# Autodesk Inventor assembly: right_leg
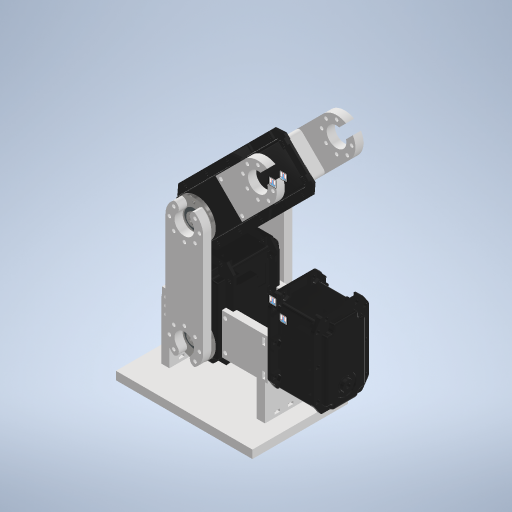
[picture p0: Inventor's stored thumbnail of the model, 512x512]
Saved by Autodesk Inventor 2024.3 (Build 283343000, 343)
## iProperties
Created: 2024-09-16
Part Number: right_leg
Document SubType Name: Assembly
Designer: USER
Author: USER
## Documents named in this file (12)
- C:\Users\USER\Desktop\로빛 예비인턴\(git)19기 이원준 격투로봇 설계파일\Lower_body\right_leg.iam
- C:\Users\USER\Desktop\로빛 예비인턴\(git)19기 이원준 격투로봇 설계파일\Lower_body\_foot.ipt
- C:\Users\USER\Desktop\로빛 예비인턴\(git)19기 이원준 격투로봇 설계파일\Lower_body\_foot_adt.ipt
- C:\Users\USER\Desktop\로빛 예비인턴\(git)19기 이원준 격투로봇 설계파일\Lower_body\_shim.ipt
- C:\Users\USER\Desktop\로빛 예비인턴\(git)19기 이원준 격투로봇 설계파일\Lower_body\_idle_adt.ipt
- C:\Users\USER\Desktop\로빛 예비인턴\(git)19기 이원준 격투로봇 설계파일\Lower_body\_adle_adt_2.ipt
- C:\Users\USER\Desktop\로빛 예비인턴\(git)19기 이원준 격투로봇 설계파일\motor\Motor_106.iam
- C:\Users\USER\Desktop\로빛 예비인턴\(git)19기 이원준 격투로봇 설계파일\아이들러\64아이들러.iam
- C:\Users\USER\Desktop\로빛 예비인턴\(git)19기 이원준 격투로봇 설계파일\motor\Motor_64_no_idle_ver.iam
- C:\Users\USER\Desktop\로빛 예비인턴\(git)19기 이원준 격투로봇 설계파일\Lower_body\_108-64_adt.ipt
- C:\Users\USER\Desktop\로빛 예비인턴\(git)19기 이원준 격투로봇 설계파일\Lower_body\_thigh.ipt
- C:\Users\USER\Desktop\로빛 예비인턴\(git)19기 이원준 격투로봇 설계파일\Lower_body\_thigh_2.ipt
## Components (18 placed, 11 different names)
1. _foot:1
2. _foot_adt:1 — 각도:2, 삽입:46, 삽입:47
3. _foot_adt:2
4. _shim:1 — 삽입:34, 삽입:36
5. _shim:2 — 삽입:35, 삽입:37, 삽입:38, 삽입:45, 각도:2
6. _idle_adt:1 — 삽입:43
7. _adle_adt_2:1
8. _idle_adt:2 — 삽입:42
9. 64아이들러:1 [sub-assembly] — 삽입:46, 삽입:47
10. Motor_64_no_idle_ver:1 [sub-assembly]
11. _108-64_adt:1 — 삽입:41
12. _108-64_adt:2 — 삽입:40
13. _thigh:1 — 삽입:31, 삽입:44
14. _thigh:2 — 삽입:29, 삽입:30, 삽입:32, 삽입:33
15. _thigh_2:1
16. _thigh_2:2
17. Motor_106:1 [sub-assembly] — 삽입:36, 삽입:37, 삽입:38, 삽입:40, 삽입:41, 삽입:42, 삽입:43
18. Motor_106:2 [sub-assembly] — 삽입:29, 삽입:30, 삽입:31, 삽입:32, 삽입:33, 삽입:34, 삽입:35, 삽입:44, 삽입:45
## Relationships (36: Insert 35, Angle 1)
- [Insert]: _foot:1 ↔ _foot_adt:1
- [Insert]: _foot:1 ↔ _foot_adt:1
- [Insert]: _foot:1 ↔ _foot_adt:2
- [Insert]: _foot:1 ↔ _foot_adt:2
- [Insert]: _adle_adt_2:1 ↔ _idle_adt:2
- [Insert]: _adle_adt_2:1 ↔ _idle_adt:2
- [Insert]: _idle_adt:1 ↔ _adle_adt_2:1
- [Insert]: _idle_adt:1 ↔ _adle_adt_2:1
- [Insert]: _foot_adt:1 ↔ 64아이들러:1
- [Insert]: _adle_adt_2:1 ↔ 64아이들러:1
- [Insert]: Motor_64_no_idle_ver:1 ↔ _108-64_adt:2
- [Insert]: Motor_64_no_idle_ver:1 ↔ _108-64_adt:2
- [Insert]: Motor_64_no_idle_ver:1 ↔ _108-64_adt:1
- [Insert]: _thigh:1 ↔ _thigh_2:1
- [Insert]: _thigh:1 ↔ _thigh_2:1
- [Insert]: _thigh:2 ↔ _thigh_2:2
- [Insert]: _thigh:2 ↔ _thigh_2:2
- 삽입:29 [Insert]: _thigh:2 ↔ Motor_106:2
- 삽입:30 [Insert]: _thigh:2 ↔ Motor_106:2
- 삽입:31 [Insert]: _thigh:1 ↔ Motor_106:2
- 삽입:32 [Insert]: _thigh:2 ↔ Motor_106:2
- 삽입:33 [Insert]: _thigh:2 ↔ Motor_106:2
- 삽입:34 [Insert]: _shim:1 ↔ Motor_106:2
- 삽입:35 [Insert]: _shim:2 ↔ Motor_106:2
- 삽입:36 [Insert]: _shim:1 ↔ Motor_106:1
- 삽입:37 [Insert]: _shim:2 ↔ Motor_106:1
- 삽입:38 [Insert]: _shim:2 ↔ Motor_106:1
- 삽입:40 [Insert]: _108-64_adt:2 ↔ Motor_106:1
- 삽입:41 [Insert]: _108-64_adt:1 ↔ Motor_106:1
- 삽입:42 [Insert]: _idle_adt:2 ↔ Motor_106:1
- 삽입:43 [Insert]: _idle_adt:1 ↔ Motor_106:1
- 삽입:44 [Insert]: _thigh:1 ↔ Motor_106:2
- 삽입:45 [Insert]: _shim:2 ↔ Motor_106:2
- 각도:2 [Angle] (0 deg): _foot_adt:1 ↔ _shim:2
- 삽입:46 [Insert]: _foot_adt:1 ↔ 64아이들러:1
- 삽입:47 [Insert]: _foot_adt:1 ↔ 64아이들러:1
